# Autodesk Inventor assembly: poot met 3 dwarsprofielen
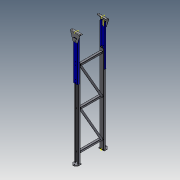
[picture p0: Inventor's stored thumbnail of the model, 180x180]
Saved by Autodesk Inventor 2015 (Build 190159000, 159)
## iProperties
Created: 2007-07-03
Part Number: poot met 3 dwarsprofielen
Document SubType Name: Assembly
Designer: kurt
Manufacturer: Standard
Standards Organization: Custom
Author: kurt
## Documents named in this file (7)
- F:\Tekeningen\bibliotheek\poten\Sub-assemblys\poot 1700-2000.iam
- F:\Tekeningen\bibliotheek\poten\onderdelen\90-08-1550.ipt
- F:\Tekeningen\bibliotheek\poten\Sub-assemblys\90-10-1550.iam
- F:\Tekeningen\bibliotheek\poten\onderdelen\90-04-0730.ipt
- F:\Tekeningen\bibliotheek\poten\onderdelen\90-09-0500.ipt
- F:\Tekeningen\bibliotheek\poten\onderdelen\90-02-0000.ipt
- F:\Tekeningen\bibliotheek\poten\onderdelen\90-03-0000.ipt
## Components (15 placed, 6 different names)
1. 90-04-0730:2 — Insert:5, Mate:17, Insert:6, Mate:18, Insert:13, Angle:1, Angle:3, Flush:10, Mate:27
2. 90-04-0730:1 — Insert:3, Insert:4, Insert:10, Insert:11, Insert:12, Flush:11
3. 90-02-0000:1 — Insert:12, Flush:8
4. 90-02-0000:2 — Insert:13, Flush:8, Angle:1
5. 90-03-0000:1 — Insert:4, Insert:11
6. 90-03-0000:2 — Insert:6, Mate:18
7. 90-03-0000:3 — Insert:5, Mate:17
8. 90-03-0000:4 — Insert:3, Insert:10, Mate:28
9. 90-10-1550:3 [sub-assembly] — Mate:22, Mate:23, Mate:24, Mate:25, Insert:14, Mate:26, Insert:15, Insert:16, Flush:9, Flush:10, Mate:27
10. 90-09-0500:1 — Mate:26, Insert:15, Insert:19
11. 90-09-0500:2 — Angle:3, Mate:25, Insert:14, Insert:17, Insert:20
12. 90-09-0500:3 — Insert:16, Flush:9, Insert:18, Flush:12
13. 90-10-1550:2 [sub-assembly] — Insert:17, Flush:11, Insert:18, Mate:28
14. 90-08-1550:1 — Flush:12
15. 90-08-1550:2 — Insert:19, Insert:20
## Relationships (31: Insert 15, Mate 9, Flush 5, Angle 2)
- Insert:3 (3 mm): 90-04-0730:1 ↔ 90-03-0000:4
- Insert:4: 90-04-0730:1 ↔ 90-03-0000:1
- Insert:5: 90-04-0730:2 ↔ 90-03-0000:3
- Mate:17: 90-04-0730:2 ↔ 90-03-0000:3
- Insert:6 (3 mm): 90-04-0730:2 ↔ 90-03-0000:2
- Mate:18: 90-04-0730:2 ↔ 90-03-0000:2
- Insert:10 (3 mm): 90-04-0730:1 ↔ 90-03-0000:4
- Insert:11: 90-04-0730:1 ↔ 90-03-0000:1
- Insert:12: 90-04-0730:1 ↔ 90-02-0000:1
- Insert:13: 90-04-0730:2 ↔ 90-02-0000:2
- Flush:8: 90-02-0000:1 ↔ 90-02-0000:2
- Angle:1 (0 deg): 90-04-0730:2 ↔ 90-02-0000:2
- Angle:3 (0 deg): 90-04-0730:2 ↔ 90-09-0500:2
- Mate:22: 90-10-1550:3
- Mate:23: 90-10-1550:3
- Mate:24: 90-10-1550:3
- Mate:25: 90-10-1550:3 ↔ 90-09-0500:2
- Insert:14 (1 mm): 90-10-1550:3 ↔ 90-09-0500:2
- Mate:26: 90-10-1550:3 ↔ 90-09-0500:1
- Insert:15 (1 mm): 90-10-1550:3 ↔ 90-09-0500:1
- Insert:16 (1 mm): 90-10-1550:3 ↔ 90-09-0500:3
- Flush:9: 90-10-1550:3 ↔ 90-09-0500:3
- Flush:10: 90-04-0730:2 ↔ 90-10-1550:3
- Mate:27: 90-04-0730:2 ↔ 90-10-1550:3
- Insert:17 (1 mm): 90-09-0500:2 ↔ 90-10-1550:2
- Flush:11: 90-04-0730:1 ↔ 90-10-1550:2
- Insert:18 (1 mm): 90-09-0500:3 ↔ 90-10-1550:2
- Mate:28: 90-03-0000:4 ↔ 90-10-1550:2
- Flush:12: 90-09-0500:3 ↔ 90-08-1550:1
- Insert:19: 90-09-0500:1 ↔ 90-08-1550:2
- Insert:20: 90-09-0500:2 ↔ 90-08-1550:2
